# Autodesk Inventor assembly: Assembly4
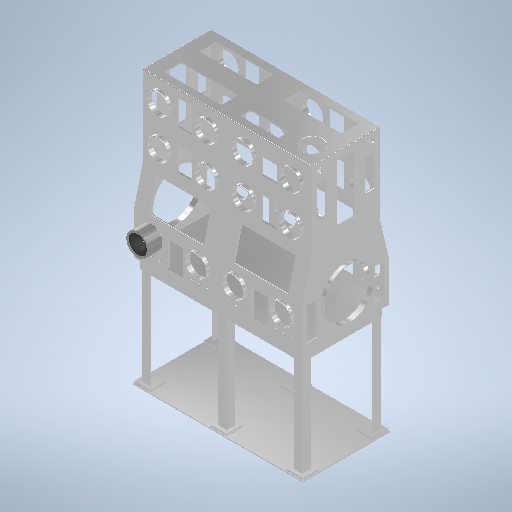
[picture p0: Inventor's stored thumbnail of the model, 512x512]
Saved by Autodesk Inventor 2025.2 (Build 292293000, 293)
## iProperties
Created: 2025-08-30
Part Number: Assembly4
Document SubType Name: Assembly
Designer: aaron
Author: aaron
## Documents named in this file (3)
- C:\Users\aaron\Documents\Inventor\Assembly4.iam
- C:\Users\aaron\Desktop\Glovebox 3D Model Updated\Glovebox 3D Model Updated\Glovebox 3D Model Updated.ipt
- C:\Users\aaron\Documents\Inventor\AirBagV1.ipt
## Components (2 placed, 2 different names)
1. Glovebox 3D Model Updated:1 — Insert:1
2. AirBagV1:1 — Insert:1
## Relationships (1: Insert 1)
- Insert:1 (-25.4 mm): Glovebox 3D Model Updated:1 ↔ AirBagV1:1
